# Autodesk Inventor assembly: nc_nhk4
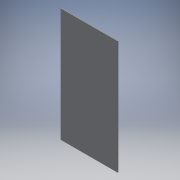
[picture p0: Inventor's stored thumbnail of the model, 180x180]
Saved by Autodesk Inventor 2019 (Build 230136000, 136)
## iProperties
Created: 2022-02-27
Part Number: nc_nhk4
Material: 一般
Document SubType Name: Assembly
Designer: yuta
Author: yuta
## Documents named in this file (4)
- C:\Users\yuta\Documents\NHK\nc_nhk4.iam
- C:\Users\yuta\Documents\NHK\NC.1.ipt
- C:\Users\yuta\Documents\NHK\nhk28.ipt
- C:\Users\yuta\Documents\NHK\nhk30.ipt
## Components (3 placed, 3 different names)
1. NC.1:1 — メイト:1, フラッシュ:1, フラッシュ:2, メイト:2, フラッシュ:3, フラッシュ:4
2. nhk28:1 — メイト:1, フラッシュ:1, フラッシュ:2
3. nhk30:1 — メイト:2, フラッシュ:3, フラッシュ:4
## Relationships (6: Flush 4, Mate 2)
- メイト:1 [Mate]: NC.1:1 ↔ nhk28:1
- フラッシュ:1 [Flush] (8 mm): NC.1:1 ↔ nhk28:1
- フラッシュ:2 [Flush] (8 mm): NC.1:1 ↔ nhk28:1
- メイト:2 [Mate]: NC.1:1 ↔ nhk30:1
- フラッシュ:3 [Flush] (8 mm): NC.1:1 ↔ nhk30:1
- フラッシュ:4 [Flush] (8 mm): NC.1:1 ↔ nhk30:1
